# Autodesk Inventor assembly: ч ASY human dummy 01
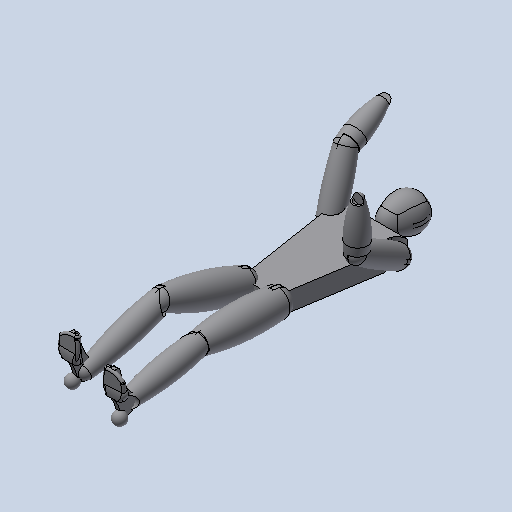
[picture p0: Inventor's stored thumbnail of the model, 512x512]
Saved by Autodesk Inventor 2025.1 (Build 291241020, 241B)
## iProperties
Created: 2018-05-21
Part Number: ч ASY human dummy 01
Material: Типовые
Document SubType Name: Assembly
Designer: admin
Stock Number: ч ASY human dummy 01
Description: Dummy
Author: admin
Revision Number: 1
## Documents named in this file (12)
- C:\Users\user\YandexDisk-badmisterfox\домашниий пк\Inventor\NDM-VOS_powder_hopper\human 01\ч ASY human dummy 01.iam
- C:\Users\user\YandexDisk-badmisterfox\домашниий пк\Inventor\NDM-VOS_powder_hopper\human 01\shoulder joint.ipt
- C:\Users\user\YandexDisk-badmisterfox\домашниий пк\Inventor\NDM-VOS_powder_hopper\human 01\Shoulder parametric.ipt
- C:\Users\user\YandexDisk-badmisterfox\домашниий пк\Inventor\NDM-VOS_powder_hopper\human 01\body parametric.ipt
- C:\Users\user\YandexDisk-badmisterfox\домашниий пк\Inventor\NDM-VOS_powder_hopper\human 01\feet parametric.ipt
- C:\Users\user\YandexDisk-badmisterfox\домашниий пк\Inventor\NDM-VOS_powder_hopper\human 01\Forearm.ipt
- C:\Users\user\YandexDisk-badmisterfox\домашниий пк\Inventor\NDM-VOS_powder_hopper\human 01\Elbow.ipt
- C:\Users\user\YandexDisk-badmisterfox\домашниий пк\Inventor\NDM-VOS_powder_hopper\human 01\Hip.ipt
- C:\Users\user\YandexDisk-badmisterfox\домашниий пк\Inventor\NDM-VOS_powder_hopper\human 01\upper leg.ipt
- C:\Users\user\YandexDisk-badmisterfox\домашниий пк\Inventor\NDM-VOS_powder_hopper\human 01\shank.ipt
- C:\Users\user\YandexDisk-badmisterfox\домашниий пк\Inventor\NDM-VOS_powder_hopper\human 01\feet parametric_MIR.ipt
- C:\Users\user\YandexDisk-badmisterfox\домашниий пк\Inventor\NDM-VOS_powder_hopper\human 01\Head.ipt
## Components (18 placed, 1 different names)
1. ч ASY human dummy 01:1 — С поворотом:1, С поворотом:9
2. ч ASY human dummy 01:2 — С поворотом:1, С поворотом:3
3. ч ASY human dummy 01:3 — Заподлицо:2, С поворотом:9, Заподлицо:7, Заподлицо:8, С поворотом:10, С поворотом:14, С поворотом:15, Совмещение:1, Заподлицо:10
4. ч ASY human dummy 01:4 — С поворотом:20
5. ч ASY human dummy 01:5 — С поворотом:2
6. ч ASY human dummy 01:6 — С поворотом:2, С поворотом:3
7. ч ASY human dummy 01:7 — С поворотом:14, С поворотом:19
8. ч ASY human dummy 01:8 — С поворотом:19, С поворотом:17
9. ч ASY human dummy 01:9 — С поворотом:18, С поворотом:16
10. ч ASY human dummy 01:10 — С поворотом:15, С поворотом:18
11. ч ASY human dummy 01:11 — С поворотом:16, С поворотом:20
12. ч ASY human dummy 01:12 — С поворотом:17, С поворотом:21
13. ч ASY human dummy 01:13 — С поворотом:10, С поворотом:11
14. ч ASY human dummy 01:14 — С поворотом:11, С поворотом:13
15. ч ASY human dummy 01:15 — С поворотом:12, С поворотом:13
16. ч ASY human dummy 01:16 — С поворотом:12
17. ч ASY human dummy 01:17 — С поворотом:21
18. ч ASY human dummy 01:18 — Заподлицо:9, Совмещение:1, Заподлицо:10
## Relationships (22: RevoluteJoint 16, Flush 5, Mate 1)
- С поворотом:1 [RevoluteJoint]: ч ASY human dummy 01:1 ↔ ч ASY human dummy 01:2
- Заподлицо:2 [Flush]: ч ASY human dummy 01:3
- С поворотом:2 [RevoluteJoint]: ч ASY human dummy 01:5 ↔ ч ASY human dummy 01:6
- С поворотом:3 [RevoluteJoint]: ч ASY human dummy 01:2 ↔ ч ASY human dummy 01:6
- С поворотом:9 [RevoluteJoint]: ч ASY human dummy 01:1 ↔ ч ASY human dummy 01:3
- Заподлицо:7 [Flush]: ч ASY human dummy 01:3
- Заподлицо:8 [Flush]: ч ASY human dummy 01:3
- С поворотом:10 [RevoluteJoint]: ч ASY human dummy 01:3 ↔ ч ASY human dummy 01:13
- С поворотом:11 [RevoluteJoint]: ч ASY human dummy 01:13 ↔ ч ASY human dummy 01:14
- С поворотом:12 [RevoluteJoint]: ч ASY human dummy 01:15 ↔ ч ASY human dummy 01:16
- С поворотом:13 [RevoluteJoint]: ч ASY human dummy 01:14 ↔ ч ASY human dummy 01:15
- С поворотом:14 [RevoluteJoint]: ч ASY human dummy 01:3 ↔ ч ASY human dummy 01:7
- С поворотом:15 [RevoluteJoint]: ч ASY human dummy 01:3 ↔ ч ASY human dummy 01:10
- С поворотом:19 [RevoluteJoint]: ч ASY human dummy 01:7 ↔ ч ASY human dummy 01:8
- С поворотом:18 [RevoluteJoint]: ч ASY human dummy 01:9 ↔ ч ASY human dummy 01:10
- С поворотом:16 [RevoluteJoint]: ч ASY human dummy 01:9 ↔ ч ASY human dummy 01:11
- С поворотом:17 [RevoluteJoint]: ч ASY human dummy 01:8 ↔ ч ASY human dummy 01:12
- С поворотом:20 [RevoluteJoint]: ч ASY human dummy 01:4 ↔ ч ASY human dummy 01:11
- С поворотом:21 [RevoluteJoint]: ч ASY human dummy 01:12 ↔ ч ASY human dummy 01:17
- Заподлицо:9 [Flush]: ч ASY human dummy 01:18
- Совмещение:1 [Mate] (100 mm): ч ASY human dummy 01:3 ↔ ч ASY human dummy 01:18
- Заподлицо:10 [Flush]: ч ASY human dummy 01:3 ↔ ч ASY human dummy 01:18
